# Autodesk Inventor assembly: Assembly3
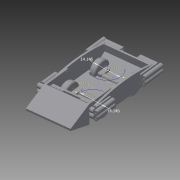
[picture p0: Inventor's stored thumbnail of the model, 180x180]
Saved by Autodesk Inventor 2015 (Build 190159000, 159)
## iProperties
Created: 2016-01-18
Part Number: Assembly3
Document SubType Name: Assembly
Designer: sethbattis
Author: sethbattis
## Documents named in this file (7)
- \\area51\team3566\cad\FRC 2016\Space Claims.iam
- \\area51\team3566\cad\FRC 2016\Basic Frame.ipt
- \\area51\team3566\cad\FRC 2016\Snow Tire Wheel with Gearbox and CIM.ipt
- \\area51\team3566\cad\FRC 2016\Corner Bumper.ipt
- \\area51\team3566\cad\FRC 2016\Wheelbase.ipt
- \\area51\team3566\cad\FRC 2016\Snow Tire Wheel with Gearbox and CIM_MIR1.ipt
- \\area51\team3566\cad\FRC 2016\Prow.ipt
## Components (11 placed, 6 different names)
1. Basic Frame:1 — Mate:7, Mate:8, Flush:4, Mate:9, Flush:5, Mate:10, Mate:11, Flush:6, Mate:12, Mate:13, Flush:7, Mate:14, Flush:8, Mate:15, Mate:16, Flush:9, Flush:10, Mate:18, Mate:19, Mate:20
2. Wheelbase:1 — Insert:1, Insert:2, Insert:3, Insert:4, Flush:10, Mate:17
3. Prow:1 — Tangent:1, Mate:18, Mate:19, Mate:20
4. Corner Bumper:1 — Mate:9, Flush:5, Mate:10, Mate:17
5. Corner Bumper:2 — Mate:11, Flush:6, Mate:12
6. Corner Bumper:3 — Mate:13, Flush:7, Mate:14
7. Corner Bumper:4 — Mate:7, Mate:8, Flush:4, Tangent:1
8. Snow Tire Wheel with Gearbox and CIM:1 — Insert:1, Flush:9
9. Snow Tire Wheel with Gearbox and CIM:2 — Insert:2, Flush:8
10. Snow Tire Wheel with Gearbox and CIM_MIR1:1 — Insert:3, Mate:15
11. Snow Tire Wheel with Gearbox and CIM_MIR1:2 — Insert:4, Mate:16
## Relationships (26: Mate 14, Flush 7, Insert 4, Tangent 1)
- Mate:7: Basic Frame:1 ↔ Corner Bumper:4
- Mate:8: Basic Frame:1 ↔ Corner Bumper:4
- Flush:4: Basic Frame:1 ↔ Corner Bumper:4
- Mate:9: Basic Frame:1 ↔ Corner Bumper:1
- Flush:5: Basic Frame:1 ↔ Corner Bumper:1
- Mate:10: Basic Frame:1 ↔ Corner Bumper:1
- Mate:11: Basic Frame:1 ↔ Corner Bumper:2
- Flush:6: Basic Frame:1 ↔ Corner Bumper:2
- Mate:12: Basic Frame:1 ↔ Corner Bumper:2
- Mate:13: Basic Frame:1 ↔ Corner Bumper:3
- Flush:7: Basic Frame:1 ↔ Corner Bumper:3
- Mate:14: Basic Frame:1 ↔ Corner Bumper:3
- Insert:1: Wheelbase:1 ↔ Snow Tire Wheel with Gearbox and CIM:1
- Insert:2: Wheelbase:1 ↔ Snow Tire Wheel with Gearbox and CIM:2
- Insert:3: Wheelbase:1 ↔ Snow Tire Wheel with Gearbox and CIM_MIR1:1
- Insert:4: Wheelbase:1 ↔ Snow Tire Wheel with Gearbox and CIM_MIR1:2
- Flush:8: Basic Frame:1 ↔ Snow Tire Wheel with Gearbox and CIM:2
- Mate:15: Basic Frame:1 ↔ Snow Tire Wheel with Gearbox and CIM_MIR1:1
- Mate:16: Basic Frame:1 ↔ Snow Tire Wheel with Gearbox and CIM_MIR1:2
- Flush:9: Basic Frame:1 ↔ Snow Tire Wheel with Gearbox and CIM:1
- Flush:10: Basic Frame:1 ↔ Wheelbase:1
- Mate:17: Wheelbase:1 ↔ Corner Bumper:1
- Tangent:1: Prow:1 ↔ Corner Bumper:4
- Mate:18: Basic Frame:1 ↔ Prow:1
- Mate:19: Basic Frame:1 ↔ Prow:1
- Mate:20: Basic Frame:1 ↔ Prow:1
